# Autodesk Inventor assembly: launcher.motor
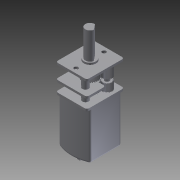
[picture p0: Inventor's stored thumbnail of the model, 180x180]
Saved by Autodesk Inventor 2011 (Build 150239000, 239)
## iProperties
Created: 2011-04-05
Part Number: launcher.motor
Document SubType Name: Assembly
Designer: Rob
Author: Rob
## Documents named in this file (5)
- C:\Users\Rob\Dropbox\RockSAT-X 2011 RexSAT\capsule-launcher.design\Launcher\launcher.motor.iam
- C:\Users\Rob\Dropbox\RockSAT-X 2011 RexSAT\capsule-launcher.design\Launcher\launcher.motor.main.ipt
- C:\Users\Rob\Dropbox\RockSAT-X 2011 RexSAT\capsule-launcher.design\Launcher\launcher.motor.shaft.ipt
- C:\Users\Rob\Dropbox\RockSAT-X 2011 RexSAT\capsule-launcher.design\Launcher\launcher.motor.midgear.ipt
- C:\Users\Rob\Dropbox\RockSAT-X 2011 RexSAT\capsule-launcher.design\Launcher\launcher.motor.lowgear.ipt
## Components (4 placed, 4 different names)
1. launcher.motor.main:1 — Mate:1, Mate:2, Mate:3, Mate:4, Mate:5, Mate:6, Mate:7
2. launcher.motor.shaft:1 — Mate:1, Mate:2, Mate:7, Rotation:1
3. launcher.motor.midgear:1 — Mate:3, Mate:4, Rotation:1, Rotation:2
4. launcher.motor.lowgear:1 — Mate:5, Mate:6, Rotation:2
## Relationships (9: Mate 7, RelateRotation 2)
- Mate:1: launcher.motor.main:1 ↔ launcher.motor.shaft:1
- Mate:2: launcher.motor.main:1 ↔ launcher.motor.shaft:1
- Mate:3: launcher.motor.main:1 ↔ launcher.motor.midgear:1
- Mate:4: launcher.motor.main:1 ↔ launcher.motor.midgear:1
- Mate:5: launcher.motor.main:1 ↔ launcher.motor.lowgear:1
- Mate:6: launcher.motor.main:1 ↔ launcher.motor.lowgear:1
- Mate:7: launcher.motor.main:1 ↔ launcher.motor.shaft:1
- Rotation:1 [RelateRotation] (2 ul): launcher.motor.shaft:1 ↔ launcher.motor.midgear:1
- Rotation:2 [RelateRotation] (0.3 ul): launcher.motor.midgear:1 ↔ launcher.motor.lowgear:1
